# Autodesk Inventor assembly: MIR_HbIndexFinger01ForChild1
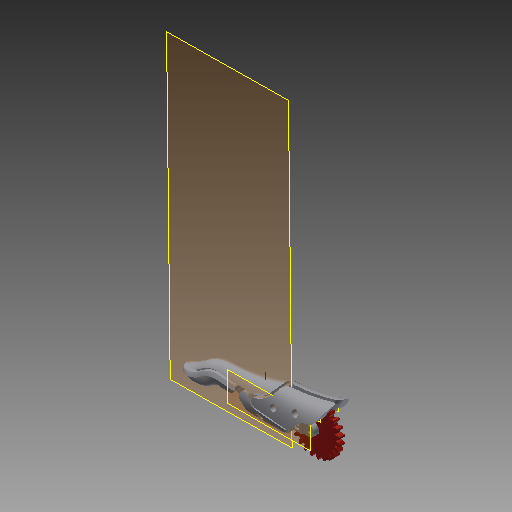
[picture p0: Inventor's stored thumbnail of the model, 512x512]
Saved by Autodesk Inventor 2018.1 (Build 221171000, 171)
## iProperties
Part Number: MIR_HbIndexFinger01ForChild1
Material: 一般
Document SubType Name: Assembly
Designer: sktom
Author: sktom
## Documents named in this file (11)
- D:\CloudStrage\OneDrive\CAD\MAJ\hackberry\HACKberry-hardware\3D_69%inlength\Inventor\HbHandForChild\HbIndexFinger01ForChild\MIR_HbIndexFinger01ForChild1.iam
- D:\CloudStrage\OneDrive\CAD\MAJ\hackberry\HACKberry-hardware\3D_69%inlength\Inventor\HbHandForChild\HbIndexFinger01ForChild\MIR_HbIndexInputLink02ForChild1.ipt
- D:\CloudStrage\OneDrive\CAD\MAJ\hackberry\HACKberry-hardware\3D_69%inlength\Inventor\HbHandForChild\HbIndexFinger01ForChild\MIR_HbIndexMiddle-DistalPhalanx02ForChild1.ipt
- D:\CloudStrage\OneDrive\CAD\MAJ\hackberry\HACKberry-hardware\3D_69%inlength\Inventor\HbHandForChild\HbIndexFinger01ForChild\MIR_HbIndexCouplerLink02ForChild1.ipt
- D:\CloudStrage\OneDrive\CAD\MAJ\hackberry\HACKberry-hardware\3D_69%inlength\Inventor\HbHandForChild\HbIndexFinger01ForChild\MIR_HbIndexCouplerLinkCover02ForChild1.ipt
- D:\CloudStrage\OneDrive\CAD\MAJ\hackberry\HACKberry-hardware\3D_69%inlength\Inventor\HbHandForChild\HbIndexFinger01ForChild\MIR_HbIndexProximalPhalanx03ForChild1.ipt
- D:\CloudStrage\OneDrive\CAD\MAJ\hackberry\HACKberry-hardware\3D_69%inlength\Inventor\HbHandForChild\HbIndexFinger01ForChild\MIR_HbIndexProximalPhalanxCover02ForChild1.ipt
- D:\CloudStrage\OneDrive\CAD\MAJ\hackberry\HACKberry-hardware\3D_69%inlength\Inventor\HbHandForChild\HbIndexFinger01ForChild\MIR_HbIndexReleaseLever02ForChild1.ipt
- D:\CloudStrage\OneDrive\CAD\MAJ\hackberry\HACKberry-hardware\3D_69%inlength\Inventor\HbHandForChild\HbIndexFinger01ForChild\MIR_Spur Gear (24 teeth)1.ipt
- D:\CloudStrage\OneDrive\CAD\MAJ\hackberry\HACKberry-hardware\3D_69%inlength\Inventor\HbHandForChild\HbIndexFinger01ForChild\MIR_shaft_phi1.5_l61.ipt
- D:\CloudStrage\OneDrive\CAD\MAJ\hackberry\HACKberry-hardware\3D_69%inlength\Inventor\HbHandForChild\MIR_TOS 0.3-3-270ﾟ-3.ipt
## Components (13 placed, 10 different names)
1. MIR_HbIndexInputLink02ForChild1:1 — 挿入:4, 円柱状:3, 円柱状:1
2. MIR_HbIndexMiddle-DistalPhalanx02ForChild1:1 — 挿入:1, 挿入:5, 円柱状:2
3. MIR_HbIndexCouplerLink02ForChild1:1 — 挿入:4, 挿入:1, 挿入:3, 挿入:2, 挿入:12, 挿入:14
4. MIR_HbIndexCouplerLinkCover02ForChild1:1 — 挿入:3, 挿入:2, 挿入:10
5. MIR_HbIndexProximalPhalanx03ForChild1:1 — 挿入:9, 円柱状:3, 円柱状:2
6. MIR_HbIndexProximalPhalanxCover02ForChild1:1 — 挿入:5, 挿入:8, 挿入:11, 挿入:13, 円柱状:1
7. MIR_HbIndexReleaseLever02ForChild1:1 — 挿入:8
8. MIR_Spur Gear (24 teeth)1:1 — 挿入:10, 挿入:9
9. MIR_shaft_phi1.5_l61:1 — 挿入:11
10. MIR_shaft_phi1.5_l61:2 — 挿入:12
11. MIR_shaft_phi1.5_l61:3 — 挿入:13
12. MIR_shaft_phi1.5_l61:4 — 挿入:14
13. MIR_TOS 0.3-3-270ﾟ-3:1
## Relationships (15: Insert 12, CylindricalJoint 3)
- 挿入:4 [Insert] (0.25 mm): MIR_HbIndexInputLink02ForChild1:1 ↔ MIR_HbIndexCouplerLink02ForChild1:1
- 挿入:1 [Insert] (0.4 mm): MIR_HbIndexMiddle-DistalPhalanx02ForChild1:1 ↔ MIR_HbIndexCouplerLink02ForChild1:1
- 挿入:3 [Insert]: MIR_HbIndexCouplerLink02ForChild1:1 ↔ MIR_HbIndexCouplerLinkCover02ForChild1:1
- 挿入:2 [Insert]: MIR_HbIndexCouplerLink02ForChild1:1 ↔ MIR_HbIndexCouplerLinkCover02ForChild1:1
- 挿入:5 [Insert] (0.4 mm): MIR_HbIndexMiddle-DistalPhalanx02ForChild1:1 ↔ MIR_HbIndexProximalPhalanxCover02ForChild1:1
- 挿入:8 [Insert] (0.2 mm): MIR_HbIndexProximalPhalanxCover02ForChild1:1 ↔ MIR_HbIndexReleaseLever02ForChild1:1
- 挿入:10 [Insert]: MIR_HbIndexCouplerLinkCover02ForChild1:1 ↔ MIR_Spur Gear (24 teeth)1:1
- 挿入:9 [Insert]: MIR_HbIndexProximalPhalanx03ForChild1:1 ↔ MIR_Spur Gear (24 teeth)1:1
- 挿入:11 [Insert] (0.5 mm): MIR_HbIndexProximalPhalanxCover02ForChild1:1 ↔ MIR_shaft_phi1.5_l61:1
- 挿入:12 [Insert] (0.5 mm): MIR_HbIndexCouplerLink02ForChild1:1 ↔ MIR_shaft_phi1.5_l61:2
- 挿入:13 [Insert] (0.5 mm): MIR_HbIndexProximalPhalanxCover02ForChild1:1 ↔ MIR_shaft_phi1.5_l61:3
- 挿入:14 [Insert] (-2 mm): MIR_HbIndexCouplerLink02ForChild1:1 ↔ MIR_shaft_phi1.5_l61:4
- 円柱状:3 [CylindricalJoint]: MIR_HbIndexInputLink02ForChild1:1 ↔ MIR_HbIndexProximalPhalanx03ForChild1:1
- 円柱状:2 [CylindricalJoint]: MIR_HbIndexMiddle-DistalPhalanx02ForChild1:1 ↔ MIR_HbIndexProximalPhalanx03ForChild1:1
- 円柱状:1 [CylindricalJoint]: MIR_HbIndexInputLink02ForChild1:1 ↔ MIR_HbIndexProximalPhalanxCover02ForChild1:1
